# Autodesk Inventor assembly: HarmonicDrive
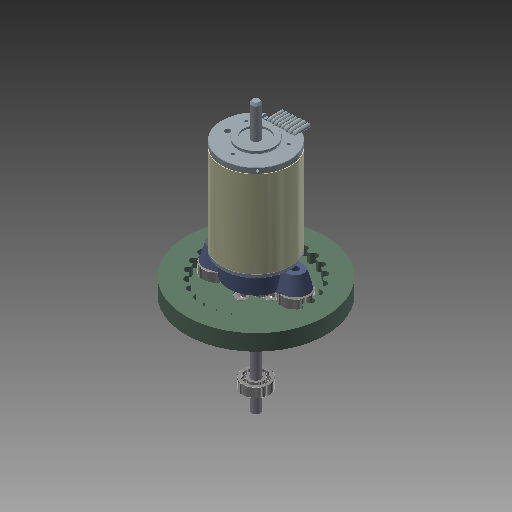
[picture p0: Inventor's stored thumbnail of the model, 512x512]
Saved by Autodesk Inventor 2018.3 (Build 223284000, 284)
## iProperties
Created: 2018-06-22
Part Number: HarmonicDrive
Material: Generisch
Document SubType Name: Assembly
Designer: JochenAlt
Author: JochenAlt
## Documents named in this file (8)
- D:\Projects\FlowerPot\CAD\HarmonicDrive.iam
- D:\Projects\FlowerPot\CAD\CircularSpline.ipt
- C:\Users\JochenAlt\Documents\Inventor\Content Center Files\R2018\de-DE\SKF - Single row ball bearings\SKF604.ipt
- D:\Projects\FlowerPot\CAD\HarmonicDrive-WaveGenerator-Bottom.ipt
- D:\Projects\FlowerPot\CAD\Mounting Hub.ipt
- D:\Projects\FlowerPot\CAD\HarmonicDrive-Axis.ipt
- C:\Users\JochenAlt\Documents\Inventor\Content Center Files\R2018\de-DE\AS 1420\AS 1420 - 1973 - M3 x 6.ipt
- D:\Projects\FlowerPot\CAD\Motor.iam
## Components (17 placed, 7 different names)
1. CircularSpline:1 — Passend:42, Passend:43, Passend:44, Passend:45, Passend:46, Passend:47, Passend:48, Passend:49, Passend:50, Passend:51
2. SKF- Kugellager, einreihig SKF604:2 — Passend:29, Passend:31, Passend:51
3. SKF- Kugellager, einreihig SKF604:1 — Passend:30, Passend:32
4. HarmonicDrive-WaveGenerator-Bottom:1 — Passend:27, Passend:28, Passend:29, Passend:30, Passend:31, Passend:32, Passend:35, Passend:37, Passend:39, Passend:41
5. Mounting Hub:1 — 0, Passend:42, Passend:52
6. HarmonicDrive-Axis:1 — 0, Passend:25, Passend:54
7. SKF- Kugellager, einreihig SKF604:3 — Passend:25, Passend:52
8. Motor:1 [sub-assembly] — Passend:27, Passend:28, Passend:34, Passend:36, Passend:38, Passend:40
9. AS 1420 - Metrisch M3 x 6:6 — Passend:34, Passend:35
10. AS 1420 - Metrisch M3 x 6:7 — Passend:36, Passend:37
11. AS 1420 - Metrisch M3 x 6:8 — Passend:38, Passend:39
12. AS 1420 - Metrisch M3 x 6:9 — Passend:40, Passend:41
13. AS 1420 - Metrisch M3 x 6:10 — Passend:43, Passend:44
14. AS 1420 - Metrisch M3 x 6:11 — Passend:45, Passend:46
15. AS 1420 - Metrisch M3 x 6:12 — Passend:47, Passend:48
16. AS 1420 - Metrisch M3 x 6:13 — Passend:49, Passend:50
17. SKF- Kugellager, einreihig SKF604:4 — Passend:54
## Relationships (28: Mate 28)
- 0 [Mate]: Mounting Hub:1 ↔ HarmonicDrive-Axis:1
- Passend:25 [Mate]: HarmonicDrive-Axis:1 ↔ SKF- Kugellager, einreihig SKF604:3
- Passend:27 [Mate]: HarmonicDrive-WaveGenerator-Bottom:1 ↔ Motor:1
- Passend:28 [Mate]: HarmonicDrive-WaveGenerator-Bottom:1 ↔ Motor:1
- Passend:29 [Mate]: SKF- Kugellager, einreihig SKF604:2 ↔ HarmonicDrive-WaveGenerator-Bottom:1
- Passend:30 [Mate]: SKF- Kugellager, einreihig SKF604:1 ↔ HarmonicDrive-WaveGenerator-Bottom:1
- Passend:31 [Mate]: SKF- Kugellager, einreihig SKF604:2 ↔ HarmonicDrive-WaveGenerator-Bottom:1
- Passend:32 [Mate]: SKF- Kugellager, einreihig SKF604:1 ↔ HarmonicDrive-WaveGenerator-Bottom:1
- Passend:34 [Mate]: Motor:1 ↔ AS 1420 - Metrisch M3 x 6:6
- Passend:35 [Mate]: HarmonicDrive-WaveGenerator-Bottom:1 ↔ AS 1420 - Metrisch M3 x 6:6
- Passend:36 [Mate]: Motor:1 ↔ AS 1420 - Metrisch M3 x 6:7
- Passend:37 [Mate]: HarmonicDrive-WaveGenerator-Bottom:1 ↔ AS 1420 - Metrisch M3 x 6:7
- Passend:38 [Mate]: Motor:1 ↔ AS 1420 - Metrisch M3 x 6:8
- Passend:39 [Mate]: HarmonicDrive-WaveGenerator-Bottom:1 ↔ AS 1420 - Metrisch M3 x 6:8
- Passend:40 [Mate]: Motor:1 ↔ AS 1420 - Metrisch M3 x 6:9
- Passend:41 [Mate]: HarmonicDrive-WaveGenerator-Bottom:1 ↔ AS 1420 - Metrisch M3 x 6:9
- Passend:42 [Mate]: CircularSpline:1 ↔ Mounting Hub:1
- Passend:43 [Mate]: CircularSpline:1 ↔ AS 1420 - Metrisch M3 x 6:10
- Passend:44 [Mate]: CircularSpline:1 ↔ AS 1420 - Metrisch M3 x 6:10
- Passend:45 [Mate]: CircularSpline:1 ↔ AS 1420 - Metrisch M3 x 6:11
- Passend:46 [Mate]: CircularSpline:1 ↔ AS 1420 - Metrisch M3 x 6:11
- Passend:47 [Mate]: CircularSpline:1 ↔ AS 1420 - Metrisch M3 x 6:12
- Passend:48 [Mate]: CircularSpline:1 ↔ AS 1420 - Metrisch M3 x 6:12
- Passend:49 [Mate]: CircularSpline:1 ↔ AS 1420 - Metrisch M3 x 6:13
- Passend:50 [Mate]: CircularSpline:1 ↔ AS 1420 - Metrisch M3 x 6:13
- Passend:51 [Mate] (0.5 mm): CircularSpline:1 ↔ SKF- Kugellager, einreihig SKF604:2
- Passend:52 [Mate]: Mounting Hub:1 ↔ SKF- Kugellager, einreihig SKF604:3
- Passend:54 [Mate]: HarmonicDrive-Axis:1 ↔ SKF- Kugellager, einreihig SKF604:4
